# Autodesk Inventor assembly: Interior Prototype
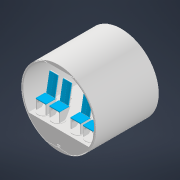
[picture p0: Inventor's stored thumbnail of the model, 180x180]
Saved by Autodesk Inventor 2021 (Build 250183000, 183)
## iProperties
Created: 2021-01-30
Part Number: Interior Prototype
Document SubType Name: Assembly
Designer: Yashipoo
Author: Yashipoo
## Documents named in this file (4)
- C:\Users\argon\OneDrive\Documents\GrabCAD\EngOne Maroons\Given Files\Interior Prototype.iam
- C:\Users\argon\OneDrive\Documents\GrabCAD\EngOne Maroons\Given Files\Tunnel.ipt
- C:\Users\argon\OneDrive\Documents\GrabCAD\EngOne Maroons\Seat Subassembly\SeatSubassembly.iam
- C:\Users\argon\OneDrive\Documents\GrabCAD\EngOne Maroons\Seat Module Subassembly\Baseplate.ipt
## Components (9 placed, 3 different names)
1. Tunnel:1 — Mate:1, Mate:2, Mate:3, Mate:7
2. SeatSubassembly:1 [sub-assembly] — Mate:4
3. SeatSubassembly:2 [sub-assembly] — Mate:5
4. SeatSubassembly:3 [sub-assembly] — Mate:6
5. SeatSubassembly:4 [sub-assembly] — Mate:8
6. Baseplate:2 — Mate:2, Mate:5
7. Baseplate:3 — Mate:1, Mate:4
8. Baseplate:4 — Mate:7, Mate:8
9. Baseplate:5 — Mate:3, Mate:6
## Relationships (8: Mate 8)
- Mate:1: Tunnel:1 ↔ Baseplate:3
- Mate:2: Tunnel:1 ↔ Baseplate:2
- Mate:3: Tunnel:1 ↔ Baseplate:5
- Mate:4: SeatSubassembly:1 ↔ Baseplate:3
- Mate:5: SeatSubassembly:2 ↔ Baseplate:2
- Mate:6: SeatSubassembly:3 ↔ Baseplate:5
- Mate:7: Tunnel:1 ↔ Baseplate:4
- Mate:8: SeatSubassembly:4 ↔ Baseplate:4
